# Autodesk Inventor assembly: BearShield
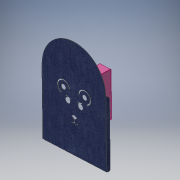
[picture p0: Inventor's stored thumbnail of the model, 180x180]
Saved by Autodesk Inventor 2019 (Build 230136000, 136)
## iProperties
Created: 2020-03-03
Part Number: BearShield
Document SubType Name: Assembly
Designer: student
Author: student
## Documents named in this file (3)
- D:\CIM\Mini-Projects\Plasma Cutter\BearShield.iam
- D:\CIM\Mini-Projects\Plasma Cutter\Handle.ipt
- D:\CIM\Mini-Projects\Plasma Cutter\Main.ipt
## Components (2 placed, 2 different names)
1. Handle:1 — Mate:2, Mate:3, Flush:2
2. Main:1 — Mate:2, Mate:3, Mate:4, Mate:5, Flush:1, Flush:2
## Relationships (6: Mate 4, Flush 2)
- Mate:2: Handle:1 ↔ Main:1
- Mate:3: Handle:1 ↔ Main:1
- Mate:4: Main:1
- Mate:5: Main:1
- Flush:1: Main:1
- Flush:2 (-31.75 mm): Handle:1 ↔ Main:1
